# Autodesk Inventor assembly: CC2x2
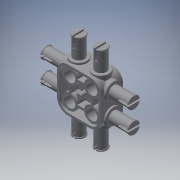
[picture p0: Inventor's stored thumbnail of the model, 180x180]
Saved by Autodesk Inventor 2019.3 (Build 233278000, 278)
## iProperties
Created: 2019-02-06
Part Number: CC2x2
Document SubType Name: Assembly
Designer: Varga Daniel
Author: Varga Daniel
## Documents named in this file (5)
- C:\!_Dani\!_cloud\OneDrive\!_munka\Revolution\RevvyDemoKit\Structural parts\Connector Boxes\Connector cubes\CC2x2.iam
- C:\!_Dani\!_cloud\OneDrive\!_munka\Revolution\RevvyDemoKit\Structural parts\Connector Boxes\Connector_box_L_base.ipt
- C:\!_Dani\!_cloud\OneDrive\!_munka\Revolution\RevvyDemoKit\Structural parts\Connector Boxes\Connector_box_collar\Connector_box_collar-one_side.ipt
- C:\!_Dani\!_cloud\OneDrive\!_munka\Revolution\RevvyDemoKit\Structural parts\Connector Boxes\Connector_box_collar.ipt
- C:\!_Dani\!_cloud\OneDrive\!_munka\Revolution\RevvyDemoKit\Structural parts\Connetor Pins\Connector_pin_stick.ipt
## Components (20 placed, 3 different names)
1. Connector_box_L_base:1 — Mate:1, Mate:2, Mate:3, Mate:4, Mate:5, Mate:6, Angle:1, Angle:2, Mate:41, Flush:1, Flush:2, Mate:43, Flush:5, Flush:6
2. Connector_box_collar-one_side:1 — Mate:4, Mate:5, Mate:6, Mate:7, Mate:8
3. Connector_box_collar-one_side:2 — Mate:1, Mate:2, Mate:3, Mate:9, Mate:10
4. Connector_pin_stick:1 — Mate:7, Mate:8, Angle:2
5. Connector_pin_stick:2 — Mate:9, Mate:10, Angle:1
6. Connector_box_L_base:2 — Mate:42, Flush:3, Flush:4
7. Connector_box_collar-one_side:3
8. Connector_box_collar-one_side:4
9. Connector_pin_stick:3
10. Connector_pin_stick:4
11. Connector_box_L_base:3 — Mate:41, Flush:1, Flush:2, Mate:42, Flush:3, Flush:4
12. Connector_box_collar-one_side:5
13. Connector_box_collar-one_side:6
14. Connector_pin_stick:5
15. Connector_pin_stick:6
16. Connector_box_L_base:4 — Mate:43, Flush:5, Flush:6
17. Connector_box_collar-one_side:7
18. Connector_box_collar-one_side:8
19. Connector_pin_stick:7
20. Connector_pin_stick:8
## Relationships (57: Mate 43, Angle 8, Flush 6)
- Mate:1: Connector_box_L_base:1 ↔ Connector_box_collar-one_side:2
- Mate:2: Connector_box_L_base:1 ↔ Connector_box_collar-one_side:2
- Mate:3: Connector_box_L_base:1 ↔ Connector_box_collar-one_side:2
- Mate:4: Connector_box_L_base:1 ↔ Connector_box_collar-one_side:1
- Mate:5: Connector_box_L_base:1 ↔ Connector_box_collar-one_side:1
- Mate:6: Connector_box_L_base:1 ↔ Connector_box_collar-one_side:1
- Mate:7: Connector_box_collar-one_side:1 ↔ Connector_pin_stick:1
- Mate:8: Connector_box_collar-one_side:1 ↔ Connector_pin_stick:1
- Mate:9: Connector_box_collar-one_side:2 ↔ Connector_pin_stick:2
- Mate:10: Connector_box_collar-one_side:2 ↔ Connector_pin_stick:2
- Angle:1 (0 deg): Connector_box_L_base:1 ↔ Connector_pin_stick:2
- Angle:2 (0 deg): Connector_box_L_base:1 ↔ Connector_pin_stick:1
- [Mate]: Connector_box_L_base:2 ↔ Connector_box_collar-one_side:4
- [Mate]: Connector_box_L_base:2 ↔ Connector_box_collar-one_side:4
- [Mate]: Connector_box_L_base:2 ↔ Connector_box_collar-one_side:4
- [Mate]: Connector_box_L_base:2 ↔ Connector_box_collar-one_side:3
- [Mate]: Connector_box_L_base:2 ↔ Connector_box_collar-one_side:3
- [Mate]: Connector_box_L_base:2 ↔ Connector_box_collar-one_side:3
- [Mate]: Connector_box_collar-one_side:3 ↔ Connector_pin_stick:3
- [Mate]: Connector_box_collar-one_side:3 ↔ Connector_pin_stick:3
- [Mate]: Connector_box_collar-one_side:4 ↔ Connector_pin_stick:4
- [Mate]: Connector_box_collar-one_side:4 ↔ Connector_pin_stick:4
- [Angle] (0 deg): Connector_box_L_base:2 ↔ Connector_pin_stick:4
- [Angle] (0 deg): Connector_box_L_base:2 ↔ Connector_pin_stick:3
- [Mate]: Connector_box_L_base:3 ↔ Connector_box_collar-one_side:6
- [Mate]: Connector_box_L_base:3 ↔ Connector_box_collar-one_side:6
- [Mate]: Connector_box_L_base:3 ↔ Connector_box_collar-one_side:6
- [Mate]: Connector_box_L_base:3 ↔ Connector_box_collar-one_side:5
- [Mate]: Connector_box_L_base:3 ↔ Connector_box_collar-one_side:5
- [Mate]: Connector_box_L_base:3 ↔ Connector_box_collar-one_side:5
- [Mate]: Connector_box_collar-one_side:5 ↔ Connector_pin_stick:5
- [Mate]: Connector_box_collar-one_side:5 ↔ Connector_pin_stick:5
- [Mate]: Connector_box_collar-one_side:6 ↔ Connector_pin_stick:6
- [Mate]: Connector_box_collar-one_side:6 ↔ Connector_pin_stick:6
- [Angle] (0 deg): Connector_box_L_base:3 ↔ Connector_pin_stick:6
- [Angle] (0 deg): Connector_box_L_base:3 ↔ Connector_pin_stick:5
- [Mate]: Connector_box_L_base:4 ↔ Connector_box_collar-one_side:8
- [Mate]: Connector_box_L_base:4 ↔ Connector_box_collar-one_side:8
- [Mate]: Connector_box_L_base:4 ↔ Connector_box_collar-one_side:8
- [Mate]: Connector_box_L_base:4 ↔ Connector_box_collar-one_side:7
- [Mate]: Connector_box_L_base:4 ↔ Connector_box_collar-one_side:7
- [Mate]: Connector_box_L_base:4 ↔ Connector_box_collar-one_side:7
- [Mate]: Connector_box_collar-one_side:7 ↔ Connector_pin_stick:7
- [Mate]: Connector_box_collar-one_side:7 ↔ Connector_pin_stick:7
- [Mate]: Connector_box_collar-one_side:8 ↔ Connector_pin_stick:8
- [Mate]: Connector_box_collar-one_side:8 ↔ Connector_pin_stick:8
- [Angle] (0 deg): Connector_box_L_base:4 ↔ Connector_pin_stick:8
- [Angle] (0 deg): Connector_box_L_base:4 ↔ Connector_pin_stick:7
- Mate:41: Connector_box_L_base:1 ↔ Connector_box_L_base:3
- Flush:1: Connector_box_L_base:1 ↔ Connector_box_L_base:3
- Flush:2: Connector_box_L_base:1 ↔ Connector_box_L_base:3
- Mate:42: Connector_box_L_base:2 ↔ Connector_box_L_base:3
- Flush:3: Connector_box_L_base:2 ↔ Connector_box_L_base:3
- Flush:4: Connector_box_L_base:2 ↔ Connector_box_L_base:3
- Mate:43: Connector_box_L_base:1 ↔ Connector_box_L_base:4
- Flush:5: Connector_box_L_base:1 ↔ Connector_box_L_base:4
- Flush:6: Connector_box_L_base:1 ↔ Connector_box_L_base:4
## Named parameters: d12_d0 = 0 mm, d13_d1 = 0 mm, d14_d2 = 0 mm, d15_d3 = 0 mm, d16_d4 = 0 mm, d17_d5 = 0 mm, d18_d6 = 0 mm, d19_d7 = 0 mm, d20_d8 = 0 mm, d21_d9 = 0 mm, d22_d10 = 0 deg, d23_d11 = 0 deg, d24_d0 = 0 mm, d25_d1 = 0 mm, d26_d2 = 0 mm, d27_d3 = 0 mm, d28_d4 = 0 mm, d29_d5 = 0 mm, d30_d6 = 0 mm, d31_d7 = 0 mm, d32_d8 = 0 mm, d33_d9 = 0 mm, d34_d10 = 0 deg, d35_d11 = 0 deg, d36_d0 = 0 mm, d37_d1 = 0 mm, d38_d2 = 0 mm, d39_d3 = 0 mm, d40_d4 = 0 mm, d41_d5 = 0 mm, d42_d6 = 0 mm, d43_d7 = 0 mm, d44_d8 = 0 mm, d45_d9 = 0 mm, d46_d10 = 0 deg, d47_d11 = 0 deg
